# Autodesk Inventor assembly: Robot Chassis 2014 Bad Arms
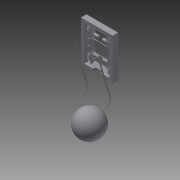
[picture p0: Inventor's stored thumbnail of the model, 180x180]
Saved by Autodesk Inventor 2013 (Build 170138000, 138)
## iProperties
Created: 2014-01-08
Part Number: Robot Chassis 2014 Bad Arms
Document SubType Name: Assembly
Designer: 300593
Translation Standard: STEP AP203
FileName: AM14U Long and AM14U Wide.STEP
PreProcessor: SolidWorks 2010
PostProcessor: Build: 138, Release: 2013 RTM - Date: Thu 03/01/2012
Sent Units: inch
Uncertainty: 1e-05
Author: 300593
## Documents named in this file (10)
- E:\Robotics\FRC\2014\CAD\Frame\Robot Chassis 2014 Bad Arms.iam
- E:\Robotics\FRC\2014\CAD\Frame\AM14U Long.iam
- E:\Robotics\FRC\2014\CAD\Frame\Left-6-inch-HD-Mecanum-Wheel.iam
- E:\Robotics\FRC\2014\CAD\Frame\Right-6-inch-HD-Mecanum-Wheel.iam
- E:\Robotics\FRC\2014\CAD\Frame\Toughbox-nano-hex-asm.iam
- E:\Robotics\FRC\2014\CAD\Additions\BumperFront.ipt
- E:\Robotics\FRC\2014\CAD\Additions\BumperSide.ipt
- E:\Robotics\FRC\2014\CAD\Additions\MammothTusk.ipt
- E:\Robotics\FRC\2014\CAD\Additions\Ball.ipt
- E:\Robotics\FRC\2014\CAD\Additions\GapBumper.ipt
## Components (16 placed, 9 different names)
1. AM14U Long:1 [sub-assembly] — Mate:1, Mate:2, Mate:3, Mate:4, Mate:5, Mate:6, Mate:7, Mate:8, Mate:9, Mate:10, Mate:11, Mate:12, Mate:17, Mate:18, Mate:19, Mate:20, Flush:1, Flush:3, Flush:5, Mate:22, Mate:26
2. Left-6-inch-HD-Mecanum-Wheel:1 [sub-assembly] — Mate:16, Mate:17
3. Left-6-inch-HD-Mecanum-Wheel:2 [sub-assembly] — Mate:14, Mate:20
4. Right-6-inch-HD-Mecanum-Wheel:1 [sub-assembly] — Mate:13, Mate:19
5. Right-6-inch-HD-Mecanum-Wheel:2 [sub-assembly] — Mate:15, Mate:18
6. Toughbox-nano-hex-asm:1 [sub-assembly] — Mate:7, Mate:10, Mate:12, Mate:13
7. Toughbox-nano-hex-asm:2 [sub-assembly] — Mate:8, Mate:9, Mate:11, Mate:14
8. Toughbox-nano-hex-asm:3 [sub-assembly] — Mate:4, Mate:5, Mate:6, Mate:15
9. Toughbox-nano-hex-asm:4 [sub-assembly] — Mate:1, Mate:2, Mate:3, Mate:16
10. BumperFront:1 — Flush:1, Flush:3, Flush:5, Flush:6, Flush:7, Flush:8, Flush:10, Flush:15
11. BumperSide:1 — Flush:6, Flush:10, Mate:29, Flush:13, Flush:14, Flush:15
12. BumperSide:2 — Mate:22, Flush:7, Flush:8
13. MammothTusk:1 — Mate:23, Flush:11, Mate:26, Flush:12, Mate:30, Mate:31
14. MammothTusk:2 — Mate:23, Flush:11, Flush:12
15. Ball:1
16. GapBumper:1 — Mate:29, Flush:13, Flush:14, Mate:30, Mate:31
## Relationships (38: Mate 26, Flush 12)
- Mate:1: AM14U Long:1 ↔ Toughbox-nano-hex-asm:4
- Mate:2: AM14U Long:1 ↔ Toughbox-nano-hex-asm:4
- Mate:3: AM14U Long:1 ↔ Toughbox-nano-hex-asm:4
- Mate:4: AM14U Long:1 ↔ Toughbox-nano-hex-asm:3
- Mate:5: AM14U Long:1 ↔ Toughbox-nano-hex-asm:3
- Mate:6: AM14U Long:1 ↔ Toughbox-nano-hex-asm:3
- Mate:7: AM14U Long:1 ↔ Toughbox-nano-hex-asm:1
- Mate:8: AM14U Long:1 ↔ Toughbox-nano-hex-asm:2
- Mate:9: AM14U Long:1 ↔ Toughbox-nano-hex-asm:2
- Mate:10: AM14U Long:1 ↔ Toughbox-nano-hex-asm:1
- Mate:11: AM14U Long:1 ↔ Toughbox-nano-hex-asm:2
- Mate:12: AM14U Long:1 ↔ Toughbox-nano-hex-asm:1
- Mate:13: Right-6-inch-HD-Mecanum-Wheel:1 ↔ Toughbox-nano-hex-asm:1
- Mate:14: Left-6-inch-HD-Mecanum-Wheel:2 ↔ Toughbox-nano-hex-asm:2
- Mate:15: Right-6-inch-HD-Mecanum-Wheel:2 ↔ Toughbox-nano-hex-asm:3
- Mate:16: Left-6-inch-HD-Mecanum-Wheel:1 ↔ Toughbox-nano-hex-asm:4
- Mate:17 (19.3294 mm): AM14U Long:1 ↔ Left-6-inch-HD-Mecanum-Wheel:1
- Mate:18 (19.3294 mm): AM14U Long:1 ↔ Right-6-inch-HD-Mecanum-Wheel:2
- Mate:19 (19.3294 mm): AM14U Long:1 ↔ Right-6-inch-HD-Mecanum-Wheel:1
- Mate:20 (19.3294 mm): AM14U Long:1 ↔ Left-6-inch-HD-Mecanum-Wheel:2
- Flush:1: AM14U Long:1 ↔ BumperFront:1
- Flush:3: AM14U Long:1 ↔ BumperFront:1
- Flush:5 (-48.3362 mm): AM14U Long:1 ↔ BumperFront:1
- Flush:6: BumperFront:1 ↔ BumperSide:1
- Mate:22: AM14U Long:1 ↔ BumperSide:2
- Flush:7: BumperFront:1 ↔ BumperSide:2
- Flush:8: BumperFront:1 ↔ BumperSide:2
- Flush:10: BumperFront:1 ↔ BumperSide:1
- Mate:23 (533.4 mm): MammothTusk:1 ↔ MammothTusk:2
- Flush:11: MammothTusk:1 ↔ MammothTusk:2
- Mate:26: AM14U Long:1 ↔ MammothTusk:1
- Flush:12: MammothTusk:1 ↔ MammothTusk:2
- Mate:29: BumperSide:1 ↔ GapBumper:1
- Flush:13: BumperSide:1 ↔ GapBumper:1
- Flush:14: BumperSide:1 ↔ GapBumper:1
- Flush:15: BumperFront:1 ↔ BumperSide:1
- Mate:30 (91.6178 mm): MammothTusk:1 ↔ GapBumper:1
- Mate:31 (25.4 mm): MammothTusk:1 ↔ GapBumper:1
